# Autodesk Inventor assembly: 機体下部
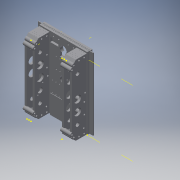
[picture p0: Inventor's stored thumbnail of the model, 180x180]
Saved by Autodesk Inventor 2018 (Build 220112000, 112)
## iProperties
Created: 2018-08-16
Part Number: 機体下部
Material: 一般
Document SubType Name: Assembly
Designer: shun2
Author: shun2
## Documents named in this file (6)
- C:\Users\shun2\OneDrive\おそらく最新版(2018.7.31)\機体下部.iam
- C:\Users\shun2\OneDrive\おそらく最新版(2018.7.31)\ギアボックス\ギアボックス片側.iam
- C:\Users\shun2\OneDrive\おそらく最新版(2018.7.31)\1枚目\一枚目.ipt
- C:\Users\shun2\OneDrive\おそらく最新版(2018.7.31)\2枚目\2枚目.ipt
- C:\Users\shun2\OneDrive\おそらく最新版(2018.7.31)\モタドラ.ipt
- C:\Users\shun2\OneDrive\おそらく最新版(2018.7.31)\基板保護2018.8.7.ipt
## Components (6 placed, 5 different names)
1. ギアボックス片側:1 [sub-assembly] — メイト:17, メイト:18, メイト:21, メイト:22
2. ギアボックス片側:2 [sub-assembly] — メイト:19, メイト:20, メイト:21, メイト:22
3. 一枚目:1 — メイト:1, メイト:3, メイト:5, メイト:6, メイト:10, メイト:11, メイト:14, メイト:15, メイト:16
4. 2枚目:1 — メイト:2, メイト:4, メイト:25, メイト:26
5. モタドラ:1 — メイト:12, メイト:13, メイト:14, メイト:15, メイト:16
6. 基板保護2018.8.7:1 — メイト:23, メイト:24
## Relationships (24: Mate 24)
- メイト:1 [Mate]: 一枚目:1
- メイト:2 [Mate]: 2枚目:1
- メイト:3 [Mate]: 一枚目:1
- メイト:4 [Mate]: 2枚目:1
- メイト:5 [Mate]: 一枚目:1
- メイト:6 [Mate]: 一枚目:1
- メイト:10 [Mate]: 一枚目:1
- メイト:11 [Mate]: 一枚目:1
- メイト:12 [Mate]: モタドラ:1
- メイト:13 [Mate]: モタドラ:1
- メイト:14 [Mate]: 一枚目:1 ↔ モタドラ:1
- メイト:15 [Mate]: 一枚目:1 ↔ モタドラ:1
- メイト:16 [Mate]: 一枚目:1 ↔ モタドラ:1
- メイト:17 [Mate]: ギアボックス片側:1
- メイト:18 [Mate]: ギアボックス片側:1
- メイト:19 [Mate]: ギアボックス片側:2
- メイト:20 [Mate]: ギアボックス片側:2
- メイト:21 [Mate]: ギアボックス片側:1 ↔ ギアボックス片側:2
- メイト:22 [Mate]: ギアボックス片側:1 ↔ ギアボックス片側:2
- メイト:23 [Mate]: 基板保護2018.8.7:1
- メイト:24 [Mate]: 基板保護2018.8.7:1
- メイト:25 [Mate]: 2枚目:1
- メイト:26 [Mate]: 2枚目:1
- メイト:27 [Mate]
